# Autodesk Inventor assembly: Body Cover Assembly
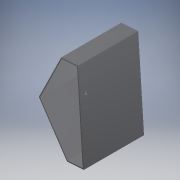
[picture p0: Inventor's stored thumbnail of the model, 180x180]
Saved by Autodesk Inventor 2017 (Build 210142000, 142)
## iProperties
Created: 2018-10-18
Part Number: Body Cover Assembly
Document SubType Name: Assembly
Designer: Dell
Author: Dell
## Documents named in this file (6)
- C:\Users\Dell\Documents\GitHub\tr2\Body\Body Cover Assembly.iam
- C:\Users\Dell\Documents\GitHub\tr2\Body\BO07.ipt
- C:\Users\Dell\Documents\GitHub\tr2\Body\BO08.ipt
- C:\Users\Dell\Documents\GitHub\tr2\Body\BO10.ipt
- C:\Users\Dell\Documents\GitHub\tr2\Body\BO11.ipt
- C:\Users\Dell\Documents\GitHub\tr2\Body\BO16.ipt
## Components (6 placed, 5 different names)
1. BO08:2 — Mate:29, Mate:33, Mate:40, Flush:6, Flush:7, Flush:12
2. BO08:3 — Mate:19, Flush:5, Mate:43, Flush:9, Flush:10
3. BO07:2 — Mate:19, Flush:5, Mate:41, Flush:8
4. BO10:1 — Mate:29, Mate:33, Mate:43, Mate:44, Flush:6, Flush:9, Flush:10, Flush:11
5. BO11:2 — Mate:44, Flush:11, Flush:12
6. BO16:1 — Mate:40, Mate:41, Flush:7, Flush:8
## Relationships (15: Flush 8, Mate 7)
- Mate:19: BO08:3 ↔ BO07:2
- Flush:5: BO08:3 ↔ BO07:2
- Mate:29: BO08:2 ↔ BO10:1
- Mate:33: BO08:2 ↔ BO10:1
- Mate:40: BO08:2 ↔ BO16:1
- Mate:41: BO07:2 ↔ BO16:1
- Mate:43: BO08:3 ↔ BO10:1
- Mate:44: BO10:1 ↔ BO11:2
- Flush:6: BO08:2 ↔ BO10:1
- Flush:7: BO08:2 ↔ BO16:1
- Flush:8: BO07:2 ↔ BO16:1
- Flush:9: BO08:3 ↔ BO10:1
- Flush:10: BO08:3 ↔ BO10:1
- Flush:11: BO10:1 ↔ BO11:2
- Flush:12: BO08:2 ↔ BO11:2
